# Autodesk Inventor assembly: CAD Model of Bridge Assembly
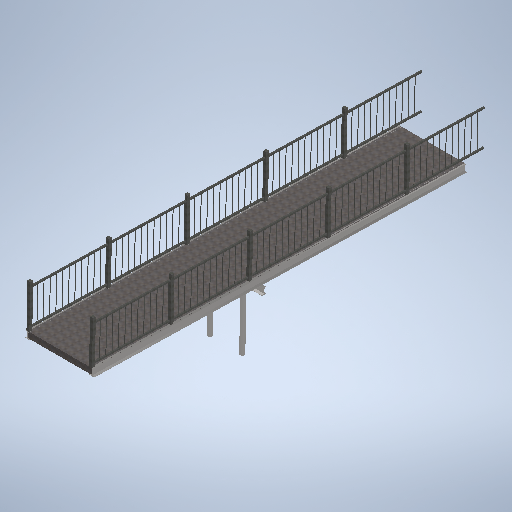
[picture p0: Inventor's stored thumbnail of the model, 512x512]
Saved by Autodesk Inventor 2025 (Build 290162000, 162)
## iProperties
Created: 2024-06-26
Part Number: CAD Model of Bridge Assembly
Document SubType Name: Assembly
Designer: track
Author: track
## Documents named in this file (7)
- C:\Users\track\OneDrive\Documents\USC-walking-bridges\Bridge_A\CAD_model\CAD Model of Bridge Assembly.iam
- C:\Users\track\OneDrive\Documents\USC-walking-bridges\Bridge_A\CAD_model\Concrete Walkway.ipt
- C:\Users\track\OneDrive\Documents\USC-walking-bridges\Bridge_A\CAD_model\Long I-Beam.ipt
- C:\Users\track\OneDrive\Documents\USC-walking-bridges\Bridge_A\CAD_model\Cylinder Supports.ipt
- C:\Users\track\OneDrive\Documents\USC-walking-bridges\Bridge_A\CAD_model\Short I-Beam.ipt
- C:\Users\track\OneDrive\Documents\USC-walking-bridges\Bridge_A\CAD_model\Railing.ipt
- C:\Users\track\OneDrive\Documents\USC-walking-bridges\Bridge_A\CAD_model\Cross Supports.ipt
## Components (16 placed, 6 different names)
1. Concrete Walkway:1 — Rigid:1, Rigid:2, Rigid:3, Mate:1, Mate:2, Flush:2, Rigid:4, Mate:7, Mate:8, Mate:9, Mate:10, Mate:11, Mate:12
2. Long I-Beam:1 — Rigid:1, Mate:3, Flush:1, Mate:4
3. Long I-Beam:2 — Rigid:2
4. Cylinder Supports:1 — Mate:5, Mate:6
5. Short I-Beam:1 — Flush:1, Mate:4, Flush:2, Mate:5, Mate:6
6. Railing:1 — Rigid:3, Rigid:5
7. Cross Supports:1 — Mate:1, Mate:2, Mate:3
8. Railing:2 — Rigid:4, Rigid:6
9. Railing:3 — Rigid:6, Rigid:8
10. Railing:4 — Mate:7, Rigid:7, Rigid:9
11. Railing:5 — Mate:8, Rigid:8, Rigid:10
12. Railing:6 — Mate:9, Rigid:11
13. Railing:7 — Rigid:5, Rigid:7
14. Railing:8 — Mate:12, Rigid:10, Rigid:12
15. Railing:9 — Mate:11, Rigid:9, Rigid:11
16. Railing:10 — Mate:10, Rigid:12
## Relationships (26: WeldJoint 12, Mate 12, Flush 2)
- Rigid:1 [WeldJoint]: Concrete Walkway:1 ↔ Long I-Beam:1
- Rigid:2 [WeldJoint]: Concrete Walkway:1 ↔ Long I-Beam:2
- Rigid:3 [WeldJoint]: Concrete Walkway:1 ↔ Railing:1
- Mate:1 (381 mm): Concrete Walkway:1 ↔ Cross Supports:1
- Mate:2: Concrete Walkway:1 ↔ Cross Supports:1
- Mate:3: Long I-Beam:1 ↔ Cross Supports:1
- Flush:1 (-120.65 mm): Long I-Beam:1 ↔ Short I-Beam:1
- Mate:4: Long I-Beam:1 ↔ Short I-Beam:1
- Flush:2 (4375.15 mm): Concrete Walkway:1 ↔ Short I-Beam:1
- Mate:5: Cylinder Supports:1 ↔ Short I-Beam:1
- Mate:6 (-533.4 mm): Cylinder Supports:1 ↔ Short I-Beam:1
- Rigid:4 [WeldJoint]: Concrete Walkway:1 ↔ Railing:2
- Rigid:5 [WeldJoint] (1981.2 mm): Railing:1 ↔ Railing:7
- Rigid:6 [WeldJoint] (1981.2 mm): Railing:2 ↔ Railing:3
- Mate:7: Concrete Walkway:1 ↔ Railing:4
- Mate:8: Concrete Walkway:1 ↔ Railing:5
- Rigid:7 [WeldJoint] (1981.2 mm): Railing:4 ↔ Railing:7
- Rigid:8 [WeldJoint] (1981.2 mm): Railing:3 ↔ Railing:5
- Mate:9: Concrete Walkway:1 ↔ Railing:6
- Mate:10: Concrete Walkway:1 ↔ Railing:10
- Mate:11: Concrete Walkway:1 ↔ Railing:9
- Mate:12: Concrete Walkway:1 ↔ Railing:8
- Rigid:9 [WeldJoint] (1981.2 mm): Railing:4 ↔ Railing:9
- Rigid:10 [WeldJoint] (1981.2 mm): Railing:5 ↔ Railing:8
- Rigid:11 [WeldJoint] (1981.2 mm): Railing:6 ↔ Railing:9
- Rigid:12 [WeldJoint] (1981.2 mm): Railing:8 ↔ Railing:10
